# Autodesk Inventor assembly: Prototipo 2
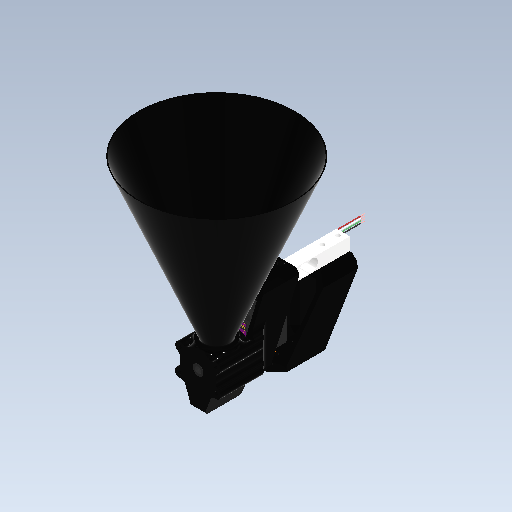
[picture p0: Inventor's stored thumbnail of the model, 512x512]
Saved by Autodesk Inventor 2020.3 (Build 243373000, 373)
## iProperties
Created: 2021-02-18
Part Number: Prototipo 2
Document SubType Name: Assembly
Designer: juanp
Author: juanp
## Documents named in this file (8)
- C:\Users\juanp\Desktop\Robocol\Nuevo EVA\V1\Dispensador\Dispensador V1.iam
- C:\Users\juanp\Desktop\Robocol\Nuevo EVA\Recursos\Servo MG996R\Servo Motor MG996R.iam
- C:\Users\juanp\Desktop\Robocol\Nuevo EVA\V1\Dispensador\attachmentcustom.ipt
- C:\Users\juanp\Desktop\Robocol\Nuevo EVA\V1\Dispensador\Valvula.ipt
- C:\Users\juanp\Desktop\Robocol\Nuevo EVA\V1\Dispensador\Retenedor.ipt
- C:\Users\juanp\Desktop\Robocol\Nuevo EVA\V1\Dispensador\Carcasa.ipt
- C:\Users\juanp\Desktop\Robocol\Nuevo EVA\Recursos\Celda de Carga\CELDA DE PRESION ARDUINO.ipt
- C:\Users\juanp\Desktop\Robocol\Nuevo EVA\V1\Dispensador\Soporte Actuador.ipt
## Components (8 placed, 7 different names)
1. Servo Motor MG996R:1 [sub-assembly] — Mate:1, Mate:2, Flush:1, Mate:3, Mate:4, Mate:11
2. attachmentcustom:1 — Mate:3, Mate:4, Mate:5, Mate:6, Flush:2, Flush:3, Mate:21, Mate:22
3. Valvula:1 — Mate:5, Mate:7, Mate:8, Mate:21
4. Retenedor:1 — Mate:6, Mate:7, Flush:2
5. Retenedor:2 — Mate:8
6. Carcasa:1 — Flush:3, Mate:11, Mate:22, Mate:23, Mate:24, Mate:25
7. CELDA DE PRESION ARDUINO:1 — Mate:23, Mate:24, Mate:25, Mate:26, Mate:27, Mate:28
8. Soporte Actuador:1 — Mate:26, Mate:27, Mate:28
## Relationships (20: Mate 17, Flush 3)
- Mate:1: Servo Motor MG996R:1
- Mate:2: Servo Motor MG996R:1
- Flush:1: Servo Motor MG996R:1
- Mate:3: Servo Motor MG996R:1 ↔ attachmentcustom:1
- Mate:4: Servo Motor MG996R:1 ↔ attachmentcustom:1
- Mate:5: attachmentcustom:1 ↔ Valvula:1
- Mate:6: attachmentcustom:1 ↔ Retenedor:1
- Mate:7: Valvula:1 ↔ Retenedor:1
- Mate:8: Valvula:1 ↔ Retenedor:2
- Flush:2 (2.5 mm): attachmentcustom:1 ↔ Retenedor:1
- Flush:3: attachmentcustom:1 ↔ Carcasa:1
- Mate:11: Servo Motor MG996R:1 ↔ Carcasa:1
- Mate:21: attachmentcustom:1 ↔ Valvula:1
- Mate:22: attachmentcustom:1 ↔ Carcasa:1
- Mate:23: Carcasa:1 ↔ CELDA DE PRESION ARDUINO:1
- Mate:24: Carcasa:1 ↔ CELDA DE PRESION ARDUINO:1
- Mate:25: Carcasa:1 ↔ CELDA DE PRESION ARDUINO:1
- Mate:26: CELDA DE PRESION ARDUINO:1 ↔ Soporte Actuador:1
- Mate:27: CELDA DE PRESION ARDUINO:1 ↔ Soporte Actuador:1
- Mate:28: CELDA DE PRESION ARDUINO:1 ↔ Soporte Actuador:1
